# Autodesk Inventor assembly: 4 Support Compartment Model 1
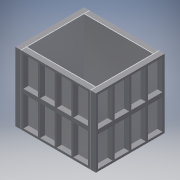
[picture p0: Inventor's stored thumbnail of the model, 180x180]
Saved by Autodesk Inventor 2017 (Build 210142000, 142)
## iProperties
Created: 2017-05-25
Part Number: 4 Support Compartment Model 1
Document SubType Name: Assembly
Designer: cas7
Author: cas7
## Documents named in this file (2)
- C:\Users\Public\Documents\Autodesk\.desktop-connect\.docstore\guided-tutorial-plugin\INVNTOR\4 Support Compartment Model 1.iam
- C:\Users\Public\Documents\Autodesk\.desktop-connect\.docstore\guided-tutorial-plugin\INVNTOR\5 Support Model.iam
## Components (8 placed, 1 different names)
1. 5 Support Model:1 [sub-assembly] — Mate:1, Mate:2, Mate:5, Mate:7
2. 5 Support Model:2 [sub-assembly] — Mate:5, Mate:6, Mate:7, Mate:15
3. 5 Support Model:3 [sub-assembly] — Mate:3, Mate:4, Mate:6, Mate:16
4. 5 Support Model:4 [sub-assembly] — Mate:1, Mate:2, Mate:3, Mate:4
5. 5 Support Model:5 [sub-assembly]
6. 5 Support Model:6 [sub-assembly] — Mate:15
7. 5 Support Model:7 [sub-assembly] — Mate:16
8. 5 Support Model:8 [sub-assembly]
## Relationships (16: Mate 16)
- Mate:1: 5 Support Model:1 ↔ 5 Support Model:4
- Mate:2: 5 Support Model:1 ↔ 5 Support Model:4
- Mate:3: 5 Support Model:3 ↔ 5 Support Model:4
- Mate:4: 5 Support Model:3 ↔ 5 Support Model:4
- Mate:5: 5 Support Model:1 ↔ 5 Support Model:2
- Mate:6: 5 Support Model:2 ↔ 5 Support Model:3
- Mate:7: 5 Support Model:1 ↔ 5 Support Model:2
- [Mate]: 5 Support Model:5 ↔ 5 Support Model:8
- [Mate]: 5 Support Model:5 ↔ 5 Support Model:8
- [Mate]: 5 Support Model:7 ↔ 5 Support Model:8
- [Mate]: 5 Support Model:7 ↔ 5 Support Model:8
- [Mate]: 5 Support Model:5 ↔ 5 Support Model:6
- [Mate]: 5 Support Model:6 ↔ 5 Support Model:7
- [Mate]: 5 Support Model:5 ↔ 5 Support Model:6
- Mate:15: 5 Support Model:2 ↔ 5 Support Model:6
- Mate:16: 5 Support Model:3 ↔ 5 Support Model:7
## Named parameters: d7_d0 = 0 mm, d8_d1 = 0 mm, d9_d2 = 0 mm, d10_d3 = 0 mm, d11_d4 = 0 mm, d12_d5 = 0 mm, d13_d6 = 0 mm
